# Autodesk Inventor assembly: 草图
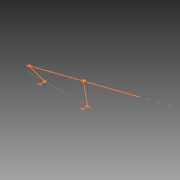
[picture p0: Inventor's stored thumbnail of the model, 180x180]
Saved by Autodesk Inventor 2011 SP2 (Build 150309200, 309)
## iProperties
Created: 2012-03-19
Part Number: 草图
Document SubType Name: Assembly
Designer: Zhensheng
Author: Zhensheng
## Documents named in this file (6)
- E:\inventor\四杆机构\草图.iam
- E:\inventor\四杆机构\草图.ipt
- E:\inventor\四杆机构\地.ipt
- E:\inventor\四杆机构\连杆1.ipt
- E:\inventor\四杆机构\连杆2.ipt
- E:\inventor\四杆机构\摇杆.ipt
## Components (5 placed, 5 different names)
1. 草图:1
2. 地:1 — 配合:1, 配合:2
3. 连杆1:1 — 配合:1, 配合:3
4. 连杆2:1 — 配合:2, 配合:4
5. 摇杆:1 — 配合:3, 配合:4
## Relationships (8: Composite 4, Mate 4)
- [Composite]: 草图:1 ↔ 地:1
- [Composite]: 草图:1 ↔ 连杆1:1
- [Composite]: 草图:1 ↔ 连杆2:1
- [Composite]: 草图:1 ↔ 摇杆:1
- 配合:1 [Mate]: 地:1 ↔ 连杆1:1
- 配合:2 [Mate]: 地:1 ↔ 连杆2:1
- 配合:3 [Mate]: 连杆1:1 ↔ 摇杆:1
- 配合:4 [Mate]: 连杆2:1 ↔ 摇杆:1
